# Autodesk Inventor assembly: MainAssembly
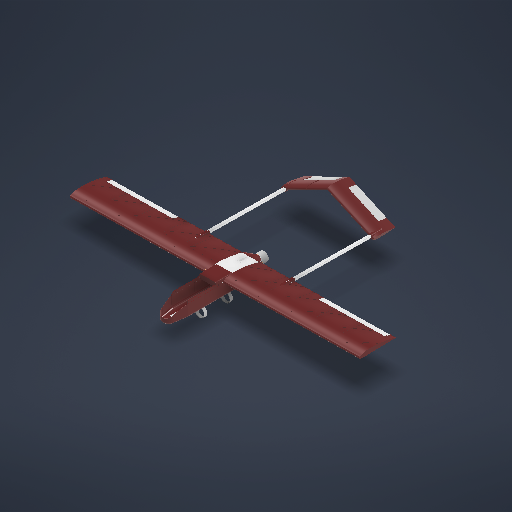
[picture p0: Inventor's stored thumbnail of the model, 512x512]
Saved by Autodesk Inventor 2026.1 (Build 301233000, 233)
## iProperties
Created: 2025-08-01
Part Number: MainAssembly
Document SubType Name: Assembly
Designer: Cupri
Author: Cupri
## Documents named in this file (19)
- C:\GitHub\SWIFT-UAV\System_development\Pelican\CAD_model\v0.2.3\MainAssembly\MainAssembly.iam
- C:\GitHub\SWIFT-UAV\System_development\Pelican\CAD_model\v0.2.3\Parts\WingParts\WingBox.ipt
- C:\GitHub\SWIFT-UAV\System_development\Pelican\CAD_model\v0.2.3\Parts\WingParts\WingLeft_v0.1.ipt
- C:\GitHub\SWIFT-UAV\System_development\Pelican\CAD_model\v0.2.3\Parts\Extrusion\20x20x1295ExtrudedAluminum.ipt
- C:\GitHub\SWIFT-UAV\System_development\Pelican\CAD_model\v0.2.3\Parts\Extrusion\20x20x800ExtrudedAluminum.ipt
- C:\GitHub\SWIFT-UAV\System_development\Pelican\CAD_model\v0.2.3\Parts\MotorHousing.ipt
- C:\GitHub\SWIFT-UAV\System_development\Pelican\CAD_model\v0.2.3\Parts\Motor.ipt
- C:\GitHub\SWIFT-UAV\System_development\Pelican\CAD_model\v0.2.3\Parts\Fueselage.ipt
- C:\GitHub\SWIFT-UAV\System_development\Pelican\CAD_model\v0.2.3\Parts\FrontCover.ipt
- C:\GitHub\SWIFT-UAV\System_development\Pelican\CAD_model\v0.2.3\Parts\AlerionLeft.ipt
- C:\GitHub\SWIFT-UAV\System_development\Pelican\CAD_model\v0.2.3\Parts\Extrusion\20x20x1295ExtrudedAluminum_MIR.ipt
- C:\GitHub\SWIFT-UAV\System_development\Pelican\CAD_model\v0.2.3\Parts\WingParts\WingLeft_v0.1_MIR1.ipt
- C:\GitHub\SWIFT-UAV\System_development\Pelican\CAD_model\v0.2.3\Parts\Extrusion\20x20x800ExtrudedAluminum_MIR2.ipt
- C:\GitHub\SWIFT-UAV\System_development\Pelican\CAD_model\v0.2.3\Parts\Tail.ipt
- C:\GitHub\SWIFT-UAV\System_development\Pelican\CAD_model\v0.2.3\Parts\Vtail.ipt
- C:\GitHub\SWIFT-UAV\System_development\Pelican\CAD_model\v0.2.3\Parts\Vtail_MIR.ipt
- C:\GitHub\SWIFT-UAV\System_development\Pelican\CAD_model\v0.2.3\Parts\AlerionLeft_MIR1.ipt
- C:\GitHub\SWIFT-UAV\System_development\Pelican\CAD_model\v0.2.3\Parts\Extrusion\20x20x785ExtrudedAluminum.ipt
- C:\GitHub\SWIFT-UAV\System_development\Pelican\CAD_model\v0.2.3\Parts\Mount v2.ipt
## Components (18 placed, 18 different names)
1. Fueselage:1 — Mate:1, Mate:2, Flush:1, Flush:7, Mate:7, Flush:11, Mate:10, Mate:11, Flush:14, Mate:23, Angle:4, Mate:27, Mate:28
2. WingBox:1 — Mate:1, Mate:2, Mate:3, Angle:1, Flush:7
3. FrontCover:1 — Flush:1
4. 20x20x1295ExtrudedAluminum:1 — Mate:4, Mate:9
5. WingLeft_v0.1:1 — Mate:5, Angle:2, Mate:7, Rotational:1
6. 20x20x800ExtrudedAluminum:1 — Mate:9, Flush:12
7. MotorHousing:1 — Flush:11, Mate:10, Mate:11, Mate:12, Mate:13, Flush:16
8. Motor:1 — Mate:12, Mate:13
9. 20x20x1295ExtrudedAluminum_MIR:1 — Mate:16, Mate:19
10. WingLeft_v0.1_MIR1:1 — Mate:18, Angle:3, Mate:20
11. 20x20x800ExtrudedAluminum_MIR2:1 — Mate:19, Mate:20
12. Tail:1 — Flush:13, Flush:14, Flush:15
13. Vtail:1 — Flush:15
14. Vtail_MIR:1
15. AlerionLeft:1 — Rotational:1
16. AlerionLeft_MIR1:1
17. 20x20x785ExtrudedAluminum:1 — Mate:26, Angle:7, Mate:29
18. Mount v2:1 — Mate:25, Angle:6, Mate:27, Mate:28, Mate:29
## Relationships (39: Mate 24, Flush 8, Angle 6, RevoluteJoint 1)
- Mate:1: Fueselage:1 ↔ WingBox:1
- Mate:2: Fueselage:1 ↔ WingBox:1
- Flush:1: Fueselage:1 ↔ FrontCover:1
- Mate:3: WingBox:1
- Angle:1 (0 deg): WingBox:1
- Mate:4: 20x20x1295ExtrudedAluminum:1
- Mate:5: WingLeft_v0.1:1
- Angle:2 (0 deg): WingLeft_v0.1:1
- Flush:7: Fueselage:1 ↔ WingBox:1
- Mate:6
- Mate:7: Fueselage:1 ↔ WingLeft_v0.1:1
- Mate:9: 20x20x1295ExtrudedAluminum:1 ↔ 20x20x800ExtrudedAluminum:1
- Flush:11: Fueselage:1 ↔ MotorHousing:1
- Mate:10: Fueselage:1 ↔ MotorHousing:1
- Mate:11: Fueselage:1 ↔ MotorHousing:1
- Mate:12: MotorHousing:1 ↔ Motor:1
- Mate:13: MotorHousing:1 ↔ Motor:1
- Mate:15
- Mate:16: 20x20x1295ExtrudedAluminum_MIR:1
- Mate:17
- Mate:18: WingLeft_v0.1_MIR1:1
- Angle:3 (0 deg): WingLeft_v0.1_MIR1:1
- Mate:19: 20x20x1295ExtrudedAluminum_MIR:1 ↔ 20x20x800ExtrudedAluminum_MIR2:1
- Mate:20: WingLeft_v0.1_MIR1:1 ↔ 20x20x800ExtrudedAluminum_MIR2:1
- Flush:12 (-100 mm): 20x20x800ExtrudedAluminum:1
- Flush:13: Tail:1
- Flush:14: Fueselage:1 ↔ Tail:1
- Flush:15: Tail:1 ↔ Vtail:1
- Mate:23: Fueselage:1
- Rotational:1 [RevoluteJoint]: WingLeft_v0.1:1 ↔ AlerionLeft:1
- Flush:16 (50 mm): MotorHousing:1
- Angle:4 (0 deg): Fueselage:1
- Mate:25: Mount v2:1
- Angle:6 (0 deg): Mount v2:1
- Mate:26: 20x20x785ExtrudedAluminum:1
- Angle:7 (0 deg): 20x20x785ExtrudedAluminum:1
- Mate:27 (0.25 mm): Fueselage:1 ↔ Mount v2:1
- Mate:28 (23 mm): Fueselage:1 ↔ Mount v2:1
- Mate:29 (0.1 mm): 20x20x785ExtrudedAluminum:1 ↔ Mount v2:1
